# Autodesk Inventor assembly: SmallSpoolAssembly
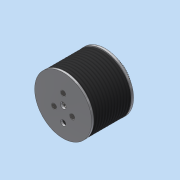
[picture p0: Inventor's stored thumbnail of the model, 180x180]
Saved by Autodesk Inventor 2017.3 (Build 213256000, 256)
## iProperties
Created: 2018-04-03
Part Number: SmallSpoolAssembly
Document SubType Name: Assembly
Designer: Derek Wider
Author: Derek Wider
## Documents named in this file (9)
- G:\Projects\Submarine\Submarine-project\CAD\midships\SpoolSection\SmallSpoolAssembly.iam
- G:\Projects\Submarine\Submarine-project\CAD\midships\SpoolSection\SmallSpoolEndAft.ipt
- G:\Projects\Submarine\Submarine-project\CAD\midships\SpoolSection\SmallSpoolEndFore.ipt
- G:\Projects\Submarine\Submarine-project\CAD\midships\SpoolSection\SpoolSmall.ipt
- G:\Projects\Submarine\Submarine-project\CAD\common\screws\flatPlasticScrewSmall.ipt
- G:\Projects\Submarine\Submarine-project\CAD\midships\SpoolSection\SpurGearLarge.ipt
- G:\Projects\Submarine\Submarine-project\CAD\common\screws\ScrewPlastic_4_20_.5inch.ipt
- G:\Projects\Submarine\Submarine-project\CAD\midships\SpoolSection\SpoolWireCoil.ipt
- G:\Projects\Submarine\Submarine-project\CAD\common\BallBearing_.25shaft_.75OD.ipt
## Components (16 placed, 8 different names)
1. SmallSpoolEndAft:1 — Mate:1, Mate:2, Mate:3, Mate:5, Flush:1, Mate:13, Mate:14, Mate:15
2. SmallSpoolEndFore:1 — Mate:4, Mate:5, Mate:6, Flush:2
3. SpoolSmall:1 — Mate:1, Mate:2, Mate:3, Mate:4, Mate:6, Mate:7, Mate:8, Mate:18, Mate:19, Flush:3, Mate:20, Flush:4
4. SpurGearLarge:1 — Mate:13, Mate:14, Mate:15, Mate:16, Mate:17
5. SpoolWireCoil:1 — Mate:18
6. BallBearing_.25shaft_.75OD:1 — Mate:19, Flush:3
7. BallBearing_.25shaft_.75OD:2 — Mate:20, Flush:4
8. flatPlasticScrewSmall:1 — Mate:7, Flush:1
9. flatPlasticScrewSmall:2
10. flatPlasticScrewSmall:3
11. flatPlasticScrewSmall:4 — Mate:8, Flush:2
12. flatPlasticScrewSmall:5
13. flatPlasticScrewSmall:6
14. ScrewPlastic_4_20_.5inch:1 — Mate:16, Mate:17
15. ScrewPlastic_4_20_.5inch:2
16. ScrewPlastic_4_20_.5inch:3
## Component patterns: (3 elements, first: flatPlasticScrewSmall:1), (3 elements, first: flatPlasticScrewSmall:4), (3 elements, first: ScrewPlastic_4_20_.5inch:1)
## Relationships (20: Mate 16, Flush 4)
- Mate:1: SmallSpoolEndAft:1 ↔ SpoolSmall:1
- Mate:2: SmallSpoolEndAft:1 ↔ SpoolSmall:1
- Mate:3: SmallSpoolEndAft:1 ↔ SpoolSmall:1
- Mate:4: SmallSpoolEndFore:1 ↔ SpoolSmall:1
- Mate:5: SmallSpoolEndAft:1 ↔ SmallSpoolEndFore:1
- Mate:6: SmallSpoolEndFore:1 ↔ SpoolSmall:1
- Mate:7: SpoolSmall:1 ↔ flatPlasticScrewSmall:1
- Flush:1: SmallSpoolEndAft:1 ↔ flatPlasticScrewSmall:1
- Mate:8: SpoolSmall:1 ↔ flatPlasticScrewSmall:4
- Flush:2: SmallSpoolEndFore:1 ↔ flatPlasticScrewSmall:4
- Mate:13: SmallSpoolEndAft:1 ↔ SpurGearLarge:1
- Mate:14: SmallSpoolEndAft:1 ↔ SpurGearLarge:1
- Mate:15: SmallSpoolEndAft:1 ↔ SpurGearLarge:1
- Mate:16: SpurGearLarge:1 ↔ ScrewPlastic_4_20_.5inch:1
- Mate:17: SpurGearLarge:1 ↔ ScrewPlastic_4_20_.5inch:1
- Mate:18: SpoolSmall:1 ↔ SpoolWireCoil:1
- Mate:19: SpoolSmall:1 ↔ BallBearing_.25shaft_.75OD:1
- Flush:3: SpoolSmall:1 ↔ BallBearing_.25shaft_.75OD:1
- Mate:20: SpoolSmall:1 ↔ BallBearing_.25shaft_.75OD:2
- Flush:4: SpoolSmall:1 ↔ BallBearing_.25shaft_.75OD:2
